# Autodesk Inventor assembly: Hing Assambly
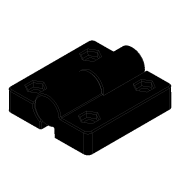
[picture p0: Inventor's stored thumbnail of the model, 180x180]
Saved by Autodesk Inventor 2015 (Build 190159000, 159)
## iProperties
Created: 2018-06-11
Part Number: Hing Assambly
Document SubType Name: Assembly
Designer: Ghassan Yusuf
Author: Ghassan Yusuf
## Documents named in this file (3)
- X:\Autodesk Designs\MakerBot Transformation\Hing Assambly.iam
- X:\Autodesk Designs\MakerBot Transformation\hing-leftSide.ipt
- X:\Autodesk Designs\MakerBot Transformation\hing-rightSide.ipt
## Components (2 placed, 2 different names)
1. hing-leftSide:1 — Insert:1, Flush:1, Insert:2
2. hing-rightSide:1 — Insert:1, Flush:1, Insert:2
## Relationships (3: Insert 2, Flush 1)
- Insert:1: hing-leftSide:1 ↔ hing-rightSide:1
- Flush:1: hing-leftSide:1 ↔ hing-rightSide:1
- Insert:2: hing-leftSide:1 ↔ hing-rightSide:1
